# Autodesk Inventor assembly: toolAssembly
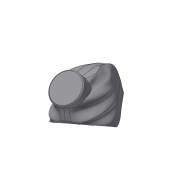
[picture p0: Inventor's stored thumbnail of the model, 180x180]
Saved by Autodesk Inventor 2018 (Build 220112000, 112)
## iProperties
Created: 2020-04-02
Part Number: toolAssembly
Document SubType Name: Assembly
Designer: Matt
Author: Matt
## Documents named in this file (5)
- C:\Users\Matt\n95\v3\formingTools\toolAssembly.iam
- C:\Users\Matt\n95\v3\formingTools\leftHalf.ipt
- C:\Users\Matt\n95\v3\formingTools\rightHalf.ipt
- C:\Users\Matt\n95\v3\formingTools\centerHalfLower.ipt
- C:\Users\Matt\n95\v3\formingTools\centerHalfUpper.ipt
## Components (4 placed, 4 different names)
1. leftHalf:1 — Mate:1, Angle:2, Flush:3, Flush:4, Flush:5
2. rightHalf:1 — Mate:1, Mate:4, Angle:1, Flush:2
3. centerHalfLower:1 — Mate:3, Flush:1, Mate:4, Angle:1, Angle:2, Flush:2, Flush:3
4. centerHalfUpper:1 — Mate:3, Flush:1, Flush:4, Flush:5
## Relationships (10: Flush 5, Mate 3, Angle 2)
- Mate:1: leftHalf:1 ↔ rightHalf:1
- Mate:3: centerHalfLower:1 ↔ centerHalfUpper:1
- Flush:1: centerHalfLower:1 ↔ centerHalfUpper:1
- Mate:4: rightHalf:1 ↔ centerHalfLower:1
- Angle:1 (0 deg): rightHalf:1 ↔ centerHalfLower:1
- Angle:2 (0 deg): leftHalf:1 ↔ centerHalfLower:1
- Flush:2 (-33.3502 mm): rightHalf:1 ↔ centerHalfLower:1
- Flush:3 (-33.3502 mm): leftHalf:1 ↔ centerHalfLower:1
- Flush:4: leftHalf:1 ↔ centerHalfUpper:1
- Flush:5: leftHalf:1 ↔ centerHalfUpper:1
